# Autodesk Inventor assembly: LegBackLinkUnitBase
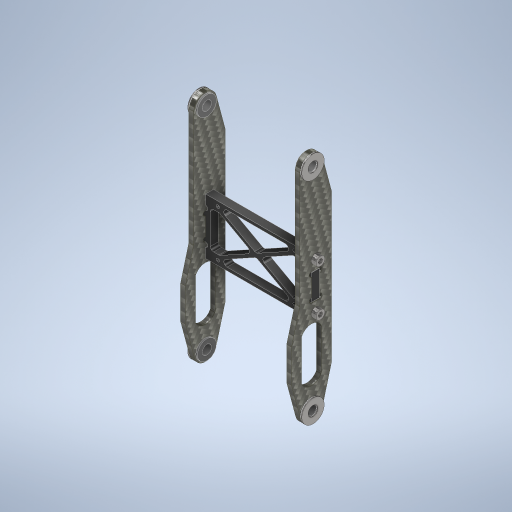
[picture p0: Inventor's stored thumbnail of the model, 512x512]
Saved by Autodesk Inventor 2024.2 (Build 282272000, 272)
## iProperties
Created: 2024-01-06
Part Number: LegBackLinkUnitBase
Document SubType Name: Assembly
Designer: Masato Kubotera
Mass: 40.5776 g
Surface Area: 239.681 cm^2
Volume: 21.0227 cm^3
Density: 1.93018 g/cm^3
Author: Masato Kubotera
## Documents named in this file (7)
- D:\OneDrive - Chiba Institute of Technology\CIT Brains\RoboCup2024\Mechanic\SUSTAINA-OP2\NativeFiles\Boby\LowerLimb\Legs\Links\LegBackLinkUnitBase.iam
- D:\OneDrive - Chiba Institute of Technology\CIT Brains\RoboCup2024\Mechanic\SUSTAINA-OP2\NativeFiles\Boby\LowerLimb\Legs\Links\LegLinkBraceFrame.ipt
- D:\OneDrive - Chiba Institute of Technology\CIT Brains\RoboCup2024\Mechanic\SUSTAINA-OP2\NativeFiles\Boby\LowerLimb\Legs\Links\LegBackLinkFrame.ipt
- D:\OneDrive - Chiba Institute of Technology\CIT Brains\RoboCup2024\Mechanic\SUSTAINA-OP2\NativeFiles\Boby\COTS\Screws\CapScrew\UC-0308.ipt
- D:\OneDrive - Chiba Institute of Technology\CIT Brains\RoboCup2024\Mechanic\SUSTAINA-OP2\NativeFiles\Boby\COTS\Bushes\GFM-0608-04.ipt
- D:\OneDrive - Chiba Institute of Technology\CIT Brains\RoboCup2024\Mechanic\SUSTAINA-OP2\NativeFiles\Boby\COTS\Washers\Resin\TT-0614-05.ipt
- D:\OneDrive - Chiba Institute of Technology\CIT Brains\RoboCup2024\Mechanic\SUSTAINA-OP2\NativeFiles\Boby\COTS\Washers\Metal\UUW-0614-05H.ipt
## Components (19 placed, 6 different names)
1. LegBackLinkFrame:1 — Insert:1, Insert:2, Insert:5, Insert:6, Insert:13, Insert:14, Insert:17, Insert:18
2. LegBackLinkFrame:2 — Insert:3, Insert:4, Insert:7, Insert:8, Insert:15, Insert:16, Insert:19, Insert:20
3. LegLinkBraceFrame:1 — Insert:1, Insert:2, Insert:3, Insert:4, Flush:1, Angle:1
4. GFM-0608-04:1 — Insert:17
5. GFM-0608-04:2 — Insert:18, Mate:1
6. GFM-0608-04:3 — Insert:19
7. GFM-0608-04:4 — Insert:20
8. UC-0308:1 — Insert:13
9. UC-0308:2 — Insert:14
10. UC-0308:3 — Insert:15
11. UC-0308:4 — Insert:16
12. TT-0614-05:4 — Insert:5, Insert:9
13. TT-0614-05:1 — Insert:6, Insert:10
14. TT-0614-05:3 — Insert:7, Insert:11
15. TT-0614-05:2 — Insert:8, Insert:12
16. UUW-0614-05H:1 — Insert:9
17. UUW-0614-05H:2 — Insert:10
18. UUW-0614-05H:3 — Insert:11
19. UUW-0614-05H:4 — Insert:12
## Relationships (23: Insert 20, Mate 1, Flush 1, Angle 1)
- Insert:1: LegBackLinkFrame:1 ↔ LegLinkBraceFrame:1
- Insert:2: LegBackLinkFrame:1 ↔ LegLinkBraceFrame:1
- Insert:3: LegBackLinkFrame:2 ↔ LegLinkBraceFrame:1
- Insert:4: LegBackLinkFrame:2 ↔ LegLinkBraceFrame:1
- Mate:1: GFM-0608-04:2
- Flush:1: LegLinkBraceFrame:1
- Angle:1 (0 deg): LegLinkBraceFrame:1
- Insert:5: LegBackLinkFrame:1 ↔ TT-0614-05:4
- Insert:6: LegBackLinkFrame:1 ↔ TT-0614-05:1
- Insert:7: LegBackLinkFrame:2 ↔ TT-0614-05:3
- Insert:8: LegBackLinkFrame:2 ↔ TT-0614-05:2
- Insert:9: TT-0614-05:4 ↔ UUW-0614-05H:1
- Insert:10: TT-0614-05:1 ↔ UUW-0614-05H:2
- Insert:11: TT-0614-05:3 ↔ UUW-0614-05H:3
- Insert:12: TT-0614-05:2 ↔ UUW-0614-05H:4
- Insert:13: LegBackLinkFrame:1 ↔ UC-0308:1
- Insert:14: LegBackLinkFrame:1 ↔ UC-0308:2
- Insert:15: LegBackLinkFrame:2 ↔ UC-0308:3
- Insert:16: LegBackLinkFrame:2 ↔ UC-0308:4
- Insert:17: LegBackLinkFrame:1 ↔ GFM-0608-04:1
- Insert:18: LegBackLinkFrame:1 ↔ GFM-0608-04:2
- Insert:19: LegBackLinkFrame:2 ↔ GFM-0608-04:3
- Insert:20: LegBackLinkFrame:2 ↔ GFM-0608-04:4
